# Autodesk Inventor assembly: MSW-13-17
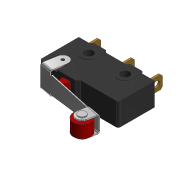
[picture p0: Inventor's stored thumbnail of the model, 180x180]
Saved by Autodesk Inventor 2014 SP2 (Build 180247200, 247)
## iProperties
Created: 2022-06-28
Part Number: MSW-13-17
Document SubType Name: Assembly
Designer: Воронежский
Mass: 1.24334 g
Surface Area: 14.062 cm^2
Volume: 1.23963 cm^3
Density: 1.00299 g/cm^3
Catalog Web Link: https://www.chipdip.ru/product/msw-13?ysclid=l57ytv4sm529010729
Vendor: «ЧИП и ДИП»
Stock Number: 493972594
TSKDver: 3.3.4.0
TSKD_DataStamp: 05.07.2022 15:29:44
Login: TAVRIDA\VPO
PCname: S-PC406
Company: ООО "Предприятие "Таврида Электрик Украина"
Mass(g): =<Mass>
TEL_ID: -
VLDS_FailCnt: 3
Author: Воронежский
Comments: MSW-13, Микропереключатель с рычагом 17 мм с роликом (5А, 125/250VAC) SPDT 3P
## Documents named in this file (5)
- D:\VaultWork\Design\Classifier\Проекты\TEU\Проекты\Для Воронежского\Workspaces\Workspace\ТЕУ ОРФС\Nomenclature group\Purchased\Electrotechnical\Микрики\MSW-13-17\MSW-13-17.iam
- MSW-13-17.iam
- D:\VaultWork\Design\Classifier\Проекты\TEU\Проекты\Для Воронежского\Workspaces\Workspace\ТЕУ ОРФС\Nomenclature group\Purchased\Electrotechnical\Микрики\MSW-13-17\MSW-13-17_body#.ipt
- D:\VaultWork\Design\Classifier\Проекты\TEU\Проекты\Для Воронежского\Workspaces\Workspace\ТЕУ ОРФС\Nomenclature group\Purchased\Electrotechnical\Микрики\MSW-13-17\MSW-13-17_button#.ipt
- D:\VaultWork\Design\Classifier\Проекты\TEU\Проекты\Для Воронежского\Workspaces\Workspace\ТЕУ ОРФС\Nomenclature group\Purchased\Electrotechnical\Микрики\MSW-13-17\MSW-13-17_lever#.ipt
## Components (3 placed, 3 different names)
1. MSW-13-17_body#:1 — Insert:1, Mate:1, Flush:1, Mate:2, Mate:3, Mate:4, Angle:1, Flush:2
2. MSW-13-17_button#:1 — Mate:2, Mate:3, Mate:4, Tangent:1
3. MSW-13-17_lever#:1 — Insert:1, Mate:1, Flush:1, Angle:1, Tangent:1
## Relationships (9: Mate 4, Flush 2, Insert 1, Angle 1, Tangent 1)
- Insert:1: MSW-13-17_body#:1 ↔ MSW-13-17_lever#:1
- Mate:1: MSW-13-17_body#:1 ↔ MSW-13-17_lever#:1
- Flush:1: MSW-13-17_body#:1 ↔ MSW-13-17_lever#:1
- Mate:2: MSW-13-17_body#:1 ↔ MSW-13-17_button#:1
- Mate:3: MSW-13-17_body#:1 ↔ MSW-13-17_button#:1
- Mate:4: MSW-13-17_body#:1 ↔ MSW-13-17_button#:1
- Angle:1 (10 deg): MSW-13-17_body#:1 ↔ MSW-13-17_lever#:1
- Flush:2: MSW-13-17_body#:1
- Tangent:1: MSW-13-17_button#:1 ↔ MSW-13-17_lever#:1
